# Autodesk Inventor assembly: coffeemakern
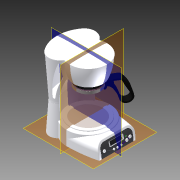
[picture p0: Inventor's stored thumbnail of the model, 180x180]
Saved by Autodesk Inventor 2015 (Build 190159000, 159)
## iProperties
Created: 2015-10-19
Part Number: coffeemakern
Document SubType Name: Assembly
Designer: omae
Author: omae
## Documents named in this file (2)
- C:\Users\omae\Desktop\研究室\論文・資料\ROS\kitchen\stl\CAD\coffeemakern.iam
- C:\Users\omae\Desktop\研究室\論文・資料\ROS\kitchen\tool\coffeemaker.iam
## Components (1 placed, 1 different names)
1. coffeemaker:1 [sub-assembly] — フラッシュ:1, フラッシュ:2, フラッシュ:3
## Relationships (3: Flush 3)
- フラッシュ:1 [Flush]: coffeemaker:1
- フラッシュ:2 [Flush]: coffeemaker:1
- フラッシュ:3 [Flush]: coffeemaker:1
